# Autodesk Inventor assembly: masbrobot 1
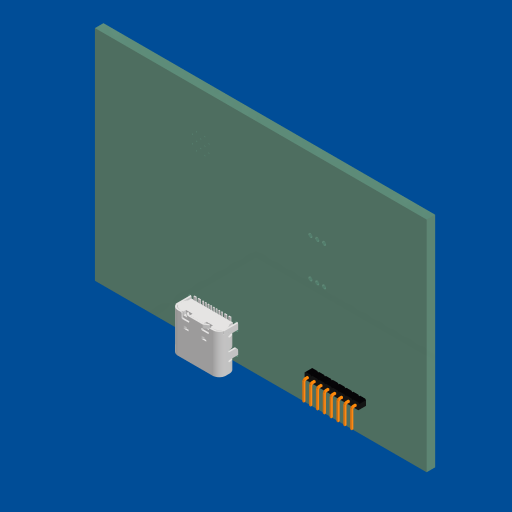
[picture p0: Inventor's stored thumbnail of the model, 512x512]
Saved by Autodesk Inventor 2023.1 (Build 271208000, 208)
## iProperties
Company: Kicad
Created: 2023-05-30
Part Number: masbrobot 1
Description: KiCad electronic assembly
Document SubType Name: Assembly
Designer: nara atthama
Authority: Unknown
Sending System: KiCad to STEP converter
Preprocessor: Open CASCADE STEP processor 7.6
Title: masbrobot.step
Author: Pcbnew
## Documents named in this file (4)
- C:\Users\naraa\OneDrive - Universitas Airlangga\Dokumen\kuliah\MATKUL\sem6\TopSus\masbrobot\model\PCB.iam
- C:\Users\naraa\OneDrive - Universitas Airlangga\Dokumen\kuliah\MATKUL\sem6\TopSus\masbrobot\model\TYPE-C-31-M-12.iam
- C:\Users\naraa\OneDrive - Universitas Airlangga\Dokumen\kuliah\MATKUL\sem6\TopSus\masbrobot\model\masbrobot PCB.ipt
- C:\Users\naraa\OneDrive - Universitas Airlangga\Dokumen\kuliah\MATKUL\sem6\TopSus\masbrobot\model\pin-header-right-male-2-54mm-1-row-1.snapshot.1\Pin header right 1 row\PinHeader_8X1_right.ipt
## Components (3 placed, 3 different names)
1. 2 [sub-assembly]
2. 3 — Mate:1
3. PinHeader_8X1_right:1 — Mate:1
## Relationships (1: Mate 1)
- Mate:1: 3 ↔ PinHeader_8X1_right:1
